# Autodesk Inventor assembly: Learnbot2
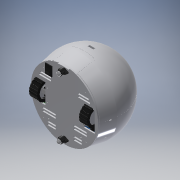
[picture p0: Inventor's stored thumbnail of the model, 180x180]
Saved by Autodesk Inventor 2017 (Build 210142000, 142)
## iProperties
Part Number: Learnbot2
Material: Genérico
Document SubType Name: Assembly
Designer: Roberto
Author: Roberto
## Documents named in this file (23)
- C:\Users\Roberto\Desktop\learnbotfinal\Learnbot2.iam
- C:\Users\Roberto\Desktop\learnbotfinal\fileToCreateTestModel\IPT\LearnbotBase.ipt
- C:\Users\Roberto\Desktop\learnbotfinal\fileToCreateTestModel\IPT\LearnbotBatteryBase.ipt
- C:\Users\Roberto\Desktop\learnbotfinal\fileToCreateTestModel\IPT\LearnbotSupportMotor.ipt
- C:\Users\Roberto\Desktop\learnbotfinal\fileToCreateTestModel\IPT\LearnbotWheel.ipt
- C:\Users\Roberto\Desktop\learnbotfinal\fileToCreateTestModel\IPT\LearnbotBattery.ipt
- C:\Users\Roberto\Desktop\learnbotfinal\fileToCreateTestModel\IPT\LearnbotCasterBall.ipt
- C:\Users\Roberto\Desktop\learnbotfinal\fileToCreateTestModel\IPT\LearnbotSupportRaspberry.ipt
- C:\Users\Roberto\Desktop\learnbotfinal\fileToCreateTestModel\IPT\LearnbotSupportLeft.ipt
- C:\Users\Roberto\Desktop\learnbotfinal\fileToCreateTestModel\IPT\LearnbotSupportRight.ipt
- C:\Users\Roberto\Desktop\learnbotfinal\fileToCreateTestModel\IPT\LearnbotServo.ipt
- C:\Users\Roberto\Desktop\learnbotfinal\fileToCreateTestModel\IPT\LearnbotPieceServo.ipt
- C:\Users\Roberto\Desktop\learnbotfinal\fileToCreateTestModel\IPT\LearnbotSupportCamera.ipt
- C:\Users\Roberto\Desktop\learnbotfinal\fileToCreateTestModel\IPT\LearnbotCamera.ipt
- C:\Users\Roberto\Desktop\learnbotfinal\fileToCreateTestModel\IPT\LearnbotSwitch.ipt
- C:\Users\Roberto\Desktop\learnbotfinal\fileToCreateTestModel\IPT\LearnbotScreen.ipt
- C:\Users\Roberto\Desktop\learnbotfinal\fileToCreateTestModel\IPT\LearnbotCoverDisplayDown.ipt
- C:\Users\Roberto\Desktop\learnbotfinal\fileToCreateTestModel\IPT\LearnbotCoverDisplayBack.ipt
- C:\Users\Roberto\Desktop\learnbotfinal\fileToCreateTestModel\IPT\LearnbotCoverDisplayUp.ipt
- C:\Users\Roberto\Desktop\learnbotfinal\fileToCreateTestModel\IPT\LearnbotFront.ipt
- C:\Users\Roberto\Desktop\learnbotfinal\fileToCreateTestModel\IPT\LearnbotLaser.ipt
- C:\Users\Roberto\Desktop\learnbotfinal\fileToCreateTestModel\IPT\LearnbotBack.ipt
- C:\Users\Roberto\Desktop\learnbotfinal\fileToCreateTestModel\IPT\LearnbotSup.ipt
## Components (32 placed, 22 different names)
1. LearnbotBase:1 — Coincidencia:1, Coincidencia:2, Coincidencia:3, Coincidencia:4, Coincidencia:9, Coincidencia:14, Coincidencia:15, Coincidencia:23, Coincidencia:24, Coincidencia:28, Coincidencia:48, Coincidencia:49
2. LearnbotBatteryBase:1 — Coincidencia:1, Coincidencia:2, Coincidencia:8, Coincidencia:12, Coincidencia:13
3. LearnbotSupportMotor:1 — Coincidencia:4, Coincidencia:5, Coincidencia:11
4. LearnbotSupportMotor:2 — Coincidencia:3, Coincidencia:6, Coincidencia:10
5. LearnbotWheel:1 — Coincidencia:5
6. LearnbotWheel:2 — Coincidencia:6
7. LearnbotCasterBall:1 — Coincidencia:8
8. LearnbotCasterBall:2 — Coincidencia:9
9. LearnbotSupportRaspberry:1 — Coincidencia:11
10. LearnbotSupportRaspberry:2 — Coincidencia:10
11. LearnbotBattery:1 — Coincidencia:12, Coincidencia:13
12. LearnbotSupportLeft:1 — Coincidencia:14, Coincidencia:25, Coincidencia:27
13. LearnbotSupportRight:1 — Coincidencia:15, Coincidencia:16, Coincidencia:17, Coincidencia:26, Coincidencia:28, Coincidencia:29
14. LearnbotServo:1 — Coincidencia:16, Coincidencia:17, Coincidencia:18, Coincidencia:19
15. LearnbotPieceServo:1 — Coincidencia:18, Coincidencia:19, Coincidencia:20, Coincidencia:21
16. LearnbotSupportCamera:1 — Coincidencia:20, Coincidencia:21, Coincidencia:22
17. LearnbotCamera:1 — Coincidencia:22
18. LearnbotSwitch:1 — Coincidencia:23, Coincidencia:24
19. LearnbotScreen:1 — Coincidencia:25, Coincidencia:26, Coincidencia:30, Coincidencia:31, Coincidencia:32
20. LearnbotCoverDisplayDown:1 — Coincidencia:27, Coincidencia:29
21. LearnbotCoverDisplayBack:1 — Coincidencia:30, Coincidencia:31, Coincidencia:32, Coincidencia:33
22. LearnbotCoverDisplayUp:1 — Coincidencia:33
23. LearnbotFront:1 — Coincidencia:34, Coincidencia:35, Coincidencia:36, Coincidencia:37, Coincidencia:38, Coincidencia:39, Coincidencia:40, Coincidencia:41, Coincidencia:42, Coincidencia:43, Coincidencia:44, Coincidencia:45, Coincidencia:46, Coincidencia:47, Coincidencia:48, Coincidencia:50
24. LearnbotLaser:1 — Coincidencia:38, Coincidencia:39
25. LearnbotLaser:2 — Coincidencia:42, Coincidencia:43
26. LearnbotLaser:3 — Coincidencia:34, Coincidencia:35
27. LearnbotLaser:4 — Coincidencia:46, Coincidencia:47
28. LearnbotLaser:5 — Coincidencia:44, Coincidencia:45
29. LearnbotLaser:6 — Coincidencia:36, Coincidencia:37
30. LearnbotLaser:7 — Coincidencia:40, Coincidencia:41
31. LearnbotBack:1 — Coincidencia:49
32. LearnbotSup:1 — Coincidencia:50
## Relationships (49: Mate 49)
- Coincidencia:1 [Mate]: LearnbotBase:1 ↔ LearnbotBatteryBase:1
- Coincidencia:2 [Mate]: LearnbotBase:1 ↔ LearnbotBatteryBase:1
- Coincidencia:3 [Mate]: LearnbotBase:1 ↔ LearnbotSupportMotor:2
- Coincidencia:4 [Mate]: LearnbotBase:1 ↔ LearnbotSupportMotor:1
- Coincidencia:5 [Mate]: LearnbotSupportMotor:1 ↔ LearnbotWheel:1
- Coincidencia:6 [Mate]: LearnbotSupportMotor:2 ↔ LearnbotWheel:2
- Coincidencia:8 [Mate]: LearnbotBatteryBase:1 ↔ LearnbotCasterBall:1
- Coincidencia:9 [Mate]: LearnbotBase:1 ↔ LearnbotCasterBall:2
- Coincidencia:10 [Mate]: LearnbotSupportMotor:2 ↔ LearnbotSupportRaspberry:2
- Coincidencia:11 [Mate]: LearnbotSupportMotor:1 ↔ LearnbotSupportRaspberry:1
- Coincidencia:12 [Mate]: LearnbotBatteryBase:1 ↔ LearnbotBattery:1
- Coincidencia:13 [Mate]: LearnbotBatteryBase:1 ↔ LearnbotBattery:1
- Coincidencia:14 [Mate]: LearnbotBase:1 ↔ LearnbotSupportLeft:1
- Coincidencia:15 [Mate]: LearnbotBase:1 ↔ LearnbotSupportRight:1
- Coincidencia:16 [Mate]: LearnbotSupportRight:1 ↔ LearnbotServo:1
- Coincidencia:17 [Mate]: LearnbotSupportRight:1 ↔ LearnbotServo:1
- Coincidencia:18 [Mate]: LearnbotServo:1 ↔ LearnbotPieceServo:1
- Coincidencia:19 [Mate]: LearnbotServo:1 ↔ LearnbotPieceServo:1
- Coincidencia:20 [Mate]: LearnbotPieceServo:1 ↔ LearnbotSupportCamera:1
- Coincidencia:21 [Mate]: LearnbotPieceServo:1 ↔ LearnbotSupportCamera:1
- Coincidencia:22 [Mate]: LearnbotSupportCamera:1 ↔ LearnbotCamera:1
- Coincidencia:23 [Mate]: LearnbotBase:1 ↔ LearnbotSwitch:1
- Coincidencia:24 [Mate]: LearnbotBase:1 ↔ LearnbotSwitch:1
- Coincidencia:25 [Mate]: LearnbotSupportLeft:1 ↔ LearnbotScreen:1
- Coincidencia:26 [Mate]: LearnbotSupportRight:1 ↔ LearnbotScreen:1
- Coincidencia:27 [Mate]: LearnbotSupportLeft:1 ↔ LearnbotCoverDisplayDown:1
- Coincidencia:28 [Mate]: LearnbotBase:1 ↔ LearnbotSupportRight:1
- Coincidencia:29 [Mate]: LearnbotSupportRight:1 ↔ LearnbotCoverDisplayDown:1
- Coincidencia:30 [Mate]: LearnbotScreen:1 ↔ LearnbotCoverDisplayBack:1
- Coincidencia:31 [Mate]: LearnbotScreen:1 ↔ LearnbotCoverDisplayBack:1
- Coincidencia:32 [Mate]: LearnbotScreen:1 ↔ LearnbotCoverDisplayBack:1
- Coincidencia:33 [Mate]: LearnbotCoverDisplayBack:1 ↔ LearnbotCoverDisplayUp:1
- Coincidencia:34 [Mate]: LearnbotFront:1 ↔ LearnbotLaser:3
- Coincidencia:35 [Mate]: LearnbotFront:1 ↔ LearnbotLaser:3
- Coincidencia:36 [Mate]: LearnbotFront:1 ↔ LearnbotLaser:6
- Coincidencia:37 [Mate]: LearnbotFront:1 ↔ LearnbotLaser:6
- Coincidencia:38 [Mate]: LearnbotFront:1 ↔ LearnbotLaser:1
- Coincidencia:39 [Mate]: LearnbotFront:1 ↔ LearnbotLaser:1
- Coincidencia:40 [Mate]: LearnbotFront:1 ↔ LearnbotLaser:7
- Coincidencia:41 [Mate]: LearnbotFront:1 ↔ LearnbotLaser:7
- Coincidencia:42 [Mate]: LearnbotFront:1 ↔ LearnbotLaser:2
- Coincidencia:43 [Mate]: LearnbotFront:1 ↔ LearnbotLaser:2
- Coincidencia:44 [Mate]: LearnbotFront:1 ↔ LearnbotLaser:5
- Coincidencia:45 [Mate]: LearnbotFront:1 ↔ LearnbotLaser:5
- Coincidencia:46 [Mate]: LearnbotFront:1 ↔ LearnbotLaser:4
- Coincidencia:47 [Mate]: LearnbotFront:1 ↔ LearnbotLaser:4
- Coincidencia:48 [Mate]: LearnbotBase:1 ↔ LearnbotFront:1
- Coincidencia:49 [Mate]: LearnbotBase:1 ↔ LearnbotBack:1
- Coincidencia:50 [Mate]: LearnbotFront:1 ↔ LearnbotSup:1
